# Autodesk Inventor assembly: Zespół14
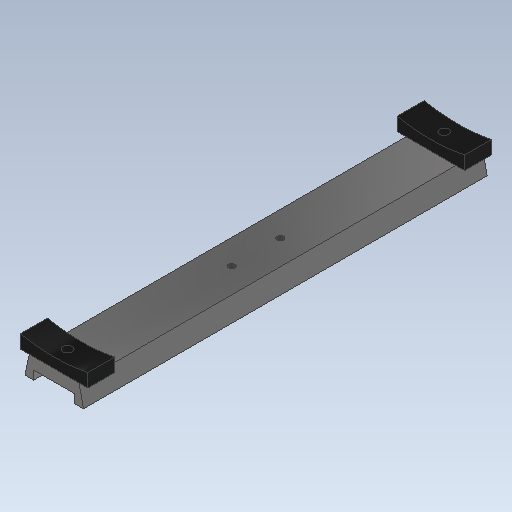
[picture p0: Inventor's stored thumbnail of the model, 512x512]
Saved by Autodesk Inventor 2020 (Build 240168000, 168)
## iProperties
Created: 2019-06-02
Part Number: Zespół14
Material: Ogólny
Document SubType Name: Assembly
Designer: barto
Author: barto
## Documents named in this file (3)
- C:\Users\Hesekiel\Desktop\Equatorial-Mount-MUM\Mechanika\Teleskop\Zespół14.iam
- C:\Users\Hesekiel\Desktop\Equatorial-Mount-MUM\Mechanika\Teleskop\szyna.ipt
- C:\Users\Hesekiel\Desktop\Equatorial-Mount-MUM\Mechanika\Teleskop\podkladka.ipt
## Components (3 placed, 2 different names)
1. szyna:1 — Zestawiające:1, Zestawiające:2, Zestawiające:3, Zestawiające:4
2. podkladka:1 — Zestawiające:2, Zestawiające:3
3. podkladka:2 — Zestawiające:1, Zestawiające:4
## Relationships (4: Mate 4)
- Zestawiające:1 [Mate]: szyna:1 ↔ podkladka:2
- Zestawiające:2 [Mate]: szyna:1 ↔ podkladka:1
- Zestawiające:3 [Mate]: szyna:1 ↔ podkladka:1
- Zestawiające:4 [Mate]: szyna:1 ↔ podkladka:2
